# Autodesk Inventor assembly: コックピット_1
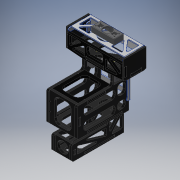
[picture p0: Inventor's stored thumbnail of the model, 180x180]
Saved by Autodesk Inventor 2018 (Build 220112000, 112)
## iProperties
Created: 2016-05-08
Part Number: コックピット_1
Document SubType Name: Assembly
Designer: hiroaki
Mass: 626.642 g
Surface Area: 2154.4 cm^2
Volume: 306.453 cm^3
Density: 2.04482 g/cm^3
Author: hiroaki
## Documents named in this file (15)
- Z:\OPR\OpenPlatform_ver1_0\上半身\コックピット\コックピット_2\コックピット_2.iam
- Z:\OPR\OpenPlatform_ver1_0\上半身\コックピット\コックピット_2\コックピット_サブフレーム_1_3.ipt
- Z:\OPR\OpenPlatform_ver1_0\上半身\コックピット\コックピット_2\コックピット_サブフレーム_1_5.ipt
- Z:\OPR\OpenPlatform_ver1_0\上半身\コックピット\コックピット_2\コックピット_サブフレーム_1_6.ipt
- Z:\OPR\OpenPlatform_ver1_0\上半身\コックピット\コックピット_2\コックピット_サブフレーム_1_7.ipt
- Z:\OPR\OpenPlatform_ver1_0\上半身\コックピット\コックピット_2\コックピット_2_メインフレーム_1.ipt
- Z:\OPR\OpenPlatform_ver1_0\上半身\コックピット\コックピット_2\コックピット_2_メインフレーム_1_MIR.ipt
- Z:\OPR\OpenPlatform_ver1_0\上半身\コックピット\コックピット_2\コックピット_2_サブフレーム_1.ipt
- Z:\OPR\OpenPlatform_ver1_0\上半身\コックピット\コックピット_2\コックピット_2_サブフレーム_2.ipt
- Z:\OPR\OpenPlatform_ver1_0\上半身\コックピット\コックピット_2\コックピット_2_サブフレーム_4.ipt
- Z:\OPR\OpenPlatform_ver1_0\上半身\コックピット\コックピット_2\コックピット_2_メインフレーム_2.ipt
- Z:\OPR\OpenPlatform_ver1_0\上半身\コックピット\コックピット_2\コックピット_2_サブフレーム_5.ipt
- Z:\OPR\OpenPlatform_ver1_0\上半身\コックピット\コックピット_2\コックピット_2_サブフレーム_6.ipt
- Z:\OPR\OpenPlatform_ver1_0\上半身\コックピット\コックピット_2\コックピット_サブフレーム_1_8.ipt
- Z:\OPR\OpenPlatform_ver1_0\既製品\sw.ipt
## Components (17 placed, 14 different names)
1. コックピット_サブフレーム_1_3:1 — 挿入:21, 挿入:22, メイト:14, メイト:15, メイト:17, メイト:19, 挿入:40, 挿入:41, 挿入:42, 挿入:43
2. コックピット_サブフレーム_1_5:1 — 挿入:21, 挿入:22, メイト:16, 挿入:24, 挿入:39
3. コックピット_サブフレーム_1_6:1 — メイト:14, メイト:15, メイト:16, メイト:18
4. コックピット_サブフレーム_1_5:2 — メイト:17, メイト:18, メイト:19, 挿入:23, 挿入:25
5. コックピット_サブフレーム_1_7:1 — 挿入:23, 挿入:24, 挿入:25, 挿入:39
6. コックピット_2_メインフレーム_1:1 — 挿入:40, 挿入:41, メイト:24, メイト:25, メイト:26, メイト:29, メイト:30, メイト:31, メイト:32, 挿入:48, 挿入:49, メイト:53, メイト:54, メイト:57, メイト:58, メイト:59
7. コックピット_2_メインフレーム_1_MIR:1 — 挿入:42, 挿入:43, メイト:27, メイト:28, メイト:33, 挿入:50, 挿入:51, 挿入:60, 挿入:61, メイト:55, メイト:56
8. コックピット_2_サブフレーム_1:1 — メイト:24, メイト:25, メイト:26, メイト:27
9. コックピット_2_サブフレーム_2:1 — メイト:28, メイト:29, メイト:30, メイト:31, メイト:32, メイト:33, 挿入:52, 挿入:53, 挿入:54, 挿入:55
10. コックピット_2_サブフレーム_4:1 — 挿入:48, 挿入:49, 挿入:50, 挿入:51
11. コックピット_2_メインフレーム_2:1 — 挿入:54, 挿入:55, メイト:44, メイト:45, 挿入:56, 挿入:57
12. コックピット_2_メインフレーム_2:2 — 挿入:52, 挿入:53, メイト:43, メイト:46, 挿入:58, 挿入:59
13. コックピット_2_サブフレーム_5:1 — メイト:43, メイト:44, メイト:45, メイト:46
14. コックピット_2_サブフレーム_6:1 — 挿入:56, 挿入:57, 挿入:58, 挿入:59
15. コックピット_サブフレーム_1_8:1 — 挿入:60, 挿入:61, メイト:53, メイト:54
16. sw:1 — メイト:55, メイト:56
17. sw:2 — メイト:57, メイト:58, メイト:59
## Relationships (51: Mate 27, Insert 24)
- 挿入:21 [Insert]: コックピット_サブフレーム_1_3:1 ↔ コックピット_サブフレーム_1_5:1
- 挿入:22 [Insert]: コックピット_サブフレーム_1_3:1 ↔ コックピット_サブフレーム_1_5:1
- メイト:14 [Mate] (0.05 mm): コックピット_サブフレーム_1_3:1 ↔ コックピット_サブフレーム_1_6:1
- メイト:15 [Mate]: コックピット_サブフレーム_1_3:1 ↔ コックピット_サブフレーム_1_6:1
- メイト:16 [Mate]: コックピット_サブフレーム_1_5:1 ↔ コックピット_サブフレーム_1_6:1
- メイト:17 [Mate]: コックピット_サブフレーム_1_3:1 ↔ コックピット_サブフレーム_1_5:2
- メイト:18 [Mate] (0.05 mm): コックピット_サブフレーム_1_6:1 ↔ コックピット_サブフレーム_1_5:2
- メイト:19 [Mate] (0.05 mm): コックピット_サブフレーム_1_3:1 ↔ コックピット_サブフレーム_1_5:2
- 挿入:23 [Insert]: コックピット_サブフレーム_1_5:2 ↔ コックピット_サブフレーム_1_7:1
- 挿入:24 [Insert]: コックピット_サブフレーム_1_5:1 ↔ コックピット_サブフレーム_1_7:1
- 挿入:25 [Insert]: コックピット_サブフレーム_1_5:2 ↔ コックピット_サブフレーム_1_7:1
- 挿入:39 [Insert]: コックピット_サブフレーム_1_5:1 ↔ コックピット_サブフレーム_1_7:1
- 挿入:40 [Insert]: コックピット_サブフレーム_1_3:1 ↔ コックピット_2_メインフレーム_1:1
- 挿入:41 [Insert]: コックピット_サブフレーム_1_3:1 ↔ コックピット_2_メインフレーム_1:1
- 挿入:42 [Insert]: コックピット_サブフレーム_1_3:1 ↔ コックピット_2_メインフレーム_1_MIR:1
- 挿入:43 [Insert]: コックピット_サブフレーム_1_3:1 ↔ コックピット_2_メインフレーム_1_MIR:1
- メイト:24 [Mate] (0.05 mm): コックピット_2_メインフレーム_1:1 ↔ コックピット_2_サブフレーム_1:1
- メイト:25 [Mate] (0.05 mm): コックピット_2_メインフレーム_1:1 ↔ コックピット_2_サブフレーム_1:1
- メイト:26 [Mate]: コックピット_2_メインフレーム_1:1 ↔ コックピット_2_サブフレーム_1:1
- メイト:27 [Mate]: コックピット_2_メインフレーム_1_MIR:1 ↔ コックピット_2_サブフレーム_1:1
- メイト:28 [Mate]: コックピット_2_メインフレーム_1_MIR:1 ↔ コックピット_2_サブフレーム_2:1
- メイト:29 [Mate]: コックピット_2_メインフレーム_1:1 ↔ コックピット_2_サブフレーム_2:1
- メイト:30 [Mate] (0.05 mm): コックピット_2_メインフレーム_1:1 ↔ コックピット_2_サブフレーム_2:1
- メイト:31 [Mate] (0.05 mm): コックピット_2_メインフレーム_1:1 ↔ コックピット_2_サブフレーム_2:1
- メイト:32 [Mate] (0.05 mm): コックピット_2_メインフレーム_1:1 ↔ コックピット_2_サブフレーム_2:1
- メイト:33 [Mate] (0.05 mm): コックピット_2_メインフレーム_1_MIR:1 ↔ コックピット_2_サブフレーム_2:1
- 挿入:48 [Insert]: コックピット_2_メインフレーム_1:1 ↔ コックピット_2_サブフレーム_4:1
- 挿入:49 [Insert]: コックピット_2_メインフレーム_1:1 ↔ コックピット_2_サブフレーム_4:1
- 挿入:50 [Insert]: コックピット_2_メインフレーム_1_MIR:1 ↔ コックピット_2_サブフレーム_4:1
- 挿入:51 [Insert]: コックピット_2_メインフレーム_1_MIR:1 ↔ コックピット_2_サブフレーム_4:1
- 挿入:52 [Insert]: コックピット_2_サブフレーム_2:1 ↔ コックピット_2_メインフレーム_2:2
- 挿入:53 [Insert]: コックピット_2_サブフレーム_2:1 ↔ コックピット_2_メインフレーム_2:2
- 挿入:54 [Insert]: コックピット_2_サブフレーム_2:1 ↔ コックピット_2_メインフレーム_2:1
- 挿入:55 [Insert]: コックピット_2_サブフレーム_2:1 ↔ コックピット_2_メインフレーム_2:1
- メイト:43 [Mate] (0.05 mm): コックピット_2_メインフレーム_2:2 ↔ コックピット_2_サブフレーム_5:1
- メイト:44 [Mate] (0.05 mm): コックピット_2_メインフレーム_2:1 ↔ コックピット_2_サブフレーム_5:1
- メイト:45 [Mate]: コックピット_2_メインフレーム_2:1 ↔ コックピット_2_サブフレーム_5:1
- メイト:46 [Mate]: コックピット_2_メインフレーム_2:2 ↔ コックピット_2_サブフレーム_5:1
- 挿入:56 [Insert]: コックピット_2_メインフレーム_2:1 ↔ コックピット_2_サブフレーム_6:1
- 挿入:57 [Insert]: コックピット_2_メインフレーム_2:1 ↔ コックピット_2_サブフレーム_6:1
- 挿入:58 [Insert]: コックピット_2_メインフレーム_2:2 ↔ コックピット_2_サブフレーム_6:1
- 挿入:59 [Insert]: コックピット_2_メインフレーム_2:2 ↔ コックピット_2_サブフレーム_6:1
- 挿入:60 [Insert]: コックピット_2_メインフレーム_1_MIR:1 ↔ コックピット_サブフレーム_1_8:1
- 挿入:61 [Insert]: コックピット_2_メインフレーム_1_MIR:1 ↔ コックピット_サブフレーム_1_8:1
- メイト:53 [Mate]: コックピット_2_メインフレーム_1:1 ↔ コックピット_サブフレーム_1_8:1
- メイト:54 [Mate]: コックピット_2_メインフレーム_1:1 ↔ コックピット_サブフレーム_1_8:1
- メイト:55 [Mate]: コックピット_2_メインフレーム_1_MIR:1 ↔ sw:1
- メイト:56 [Mate]: コックピット_2_メインフレーム_1_MIR:1 ↔ sw:1
- メイト:57 [Mate]: コックピット_2_メインフレーム_1:1 ↔ sw:2
- メイト:58 [Mate]: コックピット_2_メインフレーム_1:1 ↔ sw:2
- メイト:59 [Mate]: コックピット_2_メインフレーム_1:1 ↔ sw:2
